# Autodesk Inventor assembly: sitz_zusammenbau
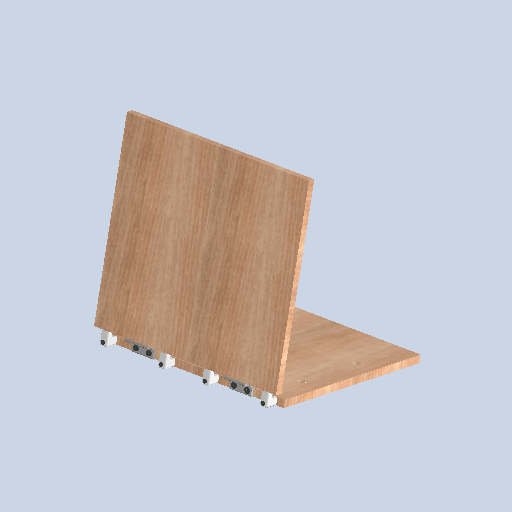
[picture p0: Inventor's stored thumbnail of the model, 512x512]
Saved by Autodesk Inventor 2024.4 (Build 284460000, 460)
## iProperties
Created: 2026-01-16
Part Number: sitz_zusammenbau
Description: Sitz_zsm
Document SubType Name: Assembly
Designer: julia
Mass: 6252.64 g
Surface Area: 11512.6 cm^2
Volume: 10145.4 cm^3
Density: 0.616304 g/cm^3
DocNumber: sitz_zusammenbau.iam
Folder: I60-Konstruktion\I60-Gruppe-7\Sitz\
VDS_Category: Konstruktion
Masse[kg]: 6,253 kg
## Documents named in this file (7)
- C:\Users\Philf\Documents\Vault\Daten\I60-Konstruktion\I60-Gruppe-7\Sitz\sitz_zusammenbau.iam
- C:\Users\Philf\Documents\Vault\Daten\I60-Konstruktion\I60-Gruppe-7\Sitz\Sitzplatte.ipt
- C:\Users\Philf\Documents\Vault\Daten\I60-Konstruktion\I60-Gruppe-7\Sitz\Sitzlehne.ipt
- C:\Users\Philf\Documents\Vault\Daten\I60-Konstruktion\I60-Gruppe-7\Sitz\Stoper.ipt
- C:\Users\Philf\Documents\Vault\Daten\I60-Konstruktion\I60-Gruppe-7\Sitz\Gelenk.iam
- C:\Users\Philf\Documents\Vault\Normteile\de-DE\ISO 10642(2)\ISO 10642  - M8  x  40.ipt
- C:\Users\Philf\Documents\Vault\Normteile\de-DE\ISO 10642(2)\ISO 10642  - M6  x  60.ipt
## Components (20 placed, 6 different names)
1. Sitzplatte:1 — Fluchtend:1, Passend:1, Fluchtend:2, Fluchtend:3, Passend:2, Fluchtend:4, Fluchtend:5, Passend:5, Fluchtend:7, Passend:6, Fluchtend:8, Fluchtend:9, Fluchtend:10, Passend:7, Passend:8, Passend:9, Passend:10, Passend:11, Passend:12, Winkel:1
2. Sitzlehne:1 — Fluchtend:5, Passend:3, Fluchtend:6, Passend:4, Winkel:1
3. Gelenk:1 [sub-assembly] — Fluchtend:1, Passend:1, Fluchtend:2, Passend:3, Fluchtend:6, Passend:13, Passend:14, Passend:21, Passend:22
4. Gelenk:2 [sub-assembly] — Fluchtend:3, Passend:2, Fluchtend:4, Passend:4, Passend:15, Passend:16, Passend:23, Passend:24
5. Stoper:1 — Passend:5, Fluchtend:7, Passend:9, Passend:20
6. Stoper:2 — Fluchtend:9, Passend:8, Passend:11, Passend:17
7. Stoper:3 — Fluchtend:10, Passend:7, Passend:10, Passend:18
8. Stoper:4 — Passend:6, Fluchtend:8, Passend:12, Passend:19
9. DIN EN ISO 10642 M8  x  40:1 — Passend:13
10. DIN EN ISO 10642 M8  x  40:2 — Passend:14
11. DIN EN ISO 10642 M8  x  40:3 — Passend:15
12. DIN EN ISO 10642 M8  x  40:4 — Passend:16
13. DIN EN ISO 10642 M6  x  60:1 — Passend:17
14. DIN EN ISO 10642 M6  x  60:2 — Passend:18
15. DIN EN ISO 10642 M6  x  60:3 — Passend:19
16. DIN EN ISO 10642 M6  x  60:4 — Passend:20
17. DIN EN ISO 10642 M8  x  40:5 — Passend:21
18. DIN EN ISO 10642 M8  x  40:6 — Passend:22
19. DIN EN ISO 10642 M8  x  40:7 — Passend:23
20. DIN EN ISO 10642 M8  x  40:8 — Passend:24
## Relationships (35: Mate 24, Flush 10, Angle 1)
- Fluchtend:1 [Flush]: Sitzplatte:1 ↔ Gelenk:1
- Passend:1 [Mate]: Sitzplatte:1 ↔ Gelenk:1
- Fluchtend:2 [Flush] (-85 mm): Sitzplatte:1 ↔ Gelenk:1
- Fluchtend:3 [Flush]: Sitzplatte:1 ↔ Gelenk:2
- Passend:2 [Mate]: Sitzplatte:1 ↔ Gelenk:2
- Fluchtend:4 [Flush] (85 mm): Sitzplatte:1 ↔ Gelenk:2
- Fluchtend:5 [Flush]: Sitzplatte:1 ↔ Sitzlehne:1
- Passend:3 [Mate]: Sitzlehne:1 ↔ Gelenk:1
- Fluchtend:6 [Flush]: Sitzlehne:1 ↔ Gelenk:1
- Passend:4 [Mate]: Sitzlehne:1 ↔ Gelenk:2
- Passend:5 [Mate]: Sitzplatte:1 ↔ Stoper:1
- Fluchtend:7 [Flush]: Sitzplatte:1 ↔ Stoper:1
- Passend:6 [Mate]: Sitzplatte:1 ↔ Stoper:4
- Fluchtend:8 [Flush]: Sitzplatte:1 ↔ Stoper:4
- Fluchtend:9 [Flush]: Sitzplatte:1 ↔ Stoper:2
- Fluchtend:10 [Flush]: Sitzplatte:1 ↔ Stoper:3
- Passend:7 [Mate]: Sitzplatte:1 ↔ Stoper:3
- Passend:8 [Mate]: Sitzplatte:1 ↔ Stoper:2
- Passend:9 [Mate] (-30 mm): Sitzplatte:1 ↔ Stoper:1
- Passend:10 [Mate] (-190 mm): Sitzplatte:1 ↔ Stoper:3
- Passend:11 [Mate] (-190 mm): Sitzplatte:1 ↔ Stoper:2
- Passend:12 [Mate] (-30 mm): Sitzplatte:1 ↔ Stoper:4
- Passend:13 [Mate]: Gelenk:1 ↔ DIN EN ISO 10642 M8  x  40:1
- Passend:14 [Mate]: Gelenk:1 ↔ DIN EN ISO 10642 M8  x  40:2
- Passend:15 [Mate]: Gelenk:2 ↔ DIN EN ISO 10642 M8  x  40:3
- Passend:16 [Mate]: Gelenk:2 ↔ DIN EN ISO 10642 M8  x  40:4
- Passend:17 [Mate]: Stoper:2 ↔ DIN EN ISO 10642 M6  x  60:1
- Passend:18 [Mate]: Stoper:3 ↔ DIN EN ISO 10642 M6  x  60:2
- Passend:19 [Mate]: Stoper:4 ↔ DIN EN ISO 10642 M6  x  60:3
- Passend:20 [Mate]: Stoper:1 ↔ DIN EN ISO 10642 M6  x  60:4
- Passend:21 [Mate]: Gelenk:1 ↔ DIN EN ISO 10642 M8  x  40:5
- Passend:22 [Mate]: Gelenk:1 ↔ DIN EN ISO 10642 M8  x  40:6
- Passend:23 [Mate]: Gelenk:2 ↔ DIN EN ISO 10642 M8  x  40:7
- Passend:24 [Mate]: Gelenk:2 ↔ DIN EN ISO 10642 M8  x  40:8
- Winkel:1 [Angle] (181 deg): Sitzplatte:1 ↔ Sitzlehne:1
